# Autodesk Inventor assembly: box assembly
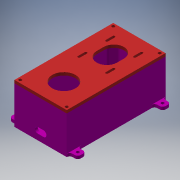
[picture p0: Inventor's stored thumbnail of the model, 180x180]
Saved by Autodesk Inventor 2018 (Build 220112000, 112)
## iProperties
Created: 2018-07-08
Part Number: box assembly
Document SubType Name: Assembly
Designer: Cole Tucker
Author: Cole Tucker
## Documents named in this file (3)
- C:\Users\Cole Tucker\OneDrive\FRC-mxpProject\Cad\sweepSensor\Inventor\v2\box assembly.iam
- C:\Users\Cole Tucker\OneDrive\FRC-mxpProject\Cad\sweepSensor\Inventor\v2\box.ipt
- C:\Users\Cole Tucker\OneDrive\FRC-mxpProject\Cad\sweepSensor\Inventor\v2\lid.ipt
## Components (2 placed, 2 different names)
1. box:1 — Mate:1, Mate:2, Mate:3
2. lid:1 — Mate:1, Mate:2, Mate:3
## Relationships (3: Mate 3)
- Mate:1: box:1 ↔ lid:1
- Mate:2: box:1 ↔ lid:1
- Mate:3: box:1 ↔ lid:1
